# Autodesk Inventor assembly: korp
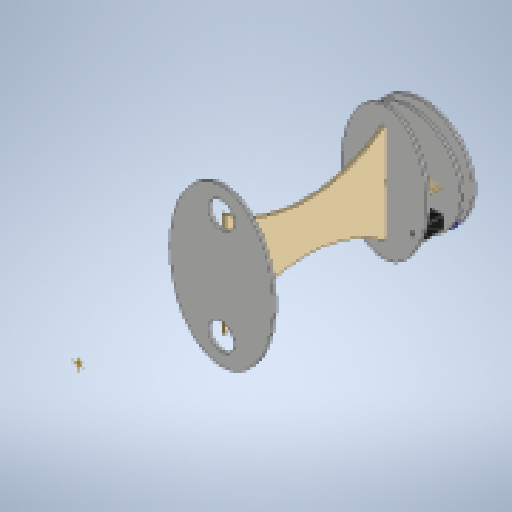
[picture p0: Inventor's stored thumbnail of the model, 512x512]
Saved by Autodesk Inventor 2023.1 (Build 271208000, 208)
## iProperties
Created: 2023-03-13
Part Number: korp
Document SubType Name: Assembly
Designer: User
Author: User
## Documents named in this file (13)
- C:\Users\DELL\reposGitHub\Cheburashka\Cheburashka_construction\korpus\korp.iam
- C:\Users\DELL\reposGitHub\Cheburashka\Cheburashka_construction\korpus\нижний эллипс тела.ipt
- C:\Users\DELL\reposGitHub\Cheburashka\Cheburashka_construction\korpus\грань тела.ipt
- C:\Users\DELL\reposGitHub\Cheburashka\Cheburashka_construction\korpus\верхний эллипс туловища.ipt
- C:\Users\DELL\reposGitHub\Cheburashka\Cheburashka_construction\korpus\нижний эллипс головы.ipt
- C:\Users\DELL\reposGitHub\Cheburashka\Cheburashka_construction\korpus\Servo.ipt
- C:\Users\DELL\reposGitHub\Cheburashka\Cheburashka_construction\korpus\крепление шеи1.ipt
- C:\Users\DELL\reposGitHub\Cheburashka\Cheburashka_construction\korpus\Pitsco Education-739028.ipt
- C:\Users\DELL\reposGitHub\Cheburashka\Cheburashka_construction\korpus\Pitsco Education-739085.ipt
- C:\Users\DELL\reposGitHub\Cheburashka\Cheburashka_construction\korpus\трубка.ipt
- C:\Users\DELL\reposGitHub\Cheburashka\Cheburashka_construction\korpus\Prostavka.ipt
- C:\Users\DELL\reposGitHub\Cheburashka\Cheburashka_construction\korpus\лицо1.ipt
- C:\Users\DELL\reposGitHub\Cheburashka\Cheburashka_construction\korpus\att_pin.ipt
## Components (13 placed, 12 different names)
1. нижний эллипс тела:1 — Заподлицо:6, Совмещение:100, Совмещение:101
2. верхний эллипс туловища:1 — Заподлицо:8, Совмещение:66, Совмещение:67, Совмещение:69
3. грань тела:1 — Заподлицо:6, Заподлицо:8, Совмещение:61, Совмещение:100, Совмещение:101
4. нижний эллипс головы:1 — Совмещение:73
5. крепление шеи1:1 — Совмещение:61
6. Pitsco Education-739028:1 — Совмещение:99
7. Pitsco Education-739085:1 — Совмещение:68, Совмещение:75, Совмещение:80
8. трубка:1 — Совмещение:66, Совмещение:67, Совмещение:68, Совмещение:74, Совмещение:81
9. Servo:4 — Совмещение:69, Совмещение:97, Совмещение:98
10. Prostavka:1 — Совмещение:73, Совмещение:74, Совмещение:75
11. Prostavka:2 — Совмещение:80, Совмещение:81, Заподлицо:16
12. лицо1:1 — Заподлицо:16
13. att_pin:1 — Совмещение:97, Совмещение:98, Совмещение:99
## Relationships (18: Mate 15, Flush 3)
- Заподлицо:6 [Flush]: нижний эллипс тела:1 ↔ грань тела:1
- Заподлицо:8 [Flush]: верхний эллипс туловища:1 ↔ грань тела:1
- Совмещение:61 [Mate]: грань тела:1 ↔ крепление шеи1:1
- Совмещение:66 [Mate]: верхний эллипс туловища:1 ↔ трубка:1
- Совмещение:67 [Mate]: верхний эллипс туловища:1 ↔ трубка:1
- Совмещение:68 [Mate]: Pitsco Education-739085:1 ↔ трубка:1
- Совмещение:69 [Mate]: верхний эллипс туловища:1 ↔ Servo:4
- Совмещение:73 [Mate]: нижний эллипс головы:1 ↔ Prostavka:1
- Совмещение:74 [Mate]: трубка:1 ↔ Prostavka:1
- Совмещение:75 [Mate]: Pitsco Education-739085:1 ↔ Prostavka:1
- Совмещение:80 [Mate]: Pitsco Education-739085:1 ↔ Prostavka:2
- Совмещение:81 [Mate]: трубка:1 ↔ Prostavka:2
- Заподлицо:16 [Flush]: Prostavka:2 ↔ лицо1:1
- Совмещение:97 [Mate]: Servo:4 ↔ att_pin:1
- Совмещение:98 [Mate]: Servo:4 ↔ att_pin:1
- Совмещение:99 [Mate]: Pitsco Education-739028:1 ↔ att_pin:1
- Совмещение:100 [Mate]: нижний эллипс тела:1 ↔ грань тела:1
- Совмещение:101 [Mate]: нижний эллипс тела:1 ↔ грань тела:1
